# Autodesk Inventor assembly: Butterfly Drive Module_MIR
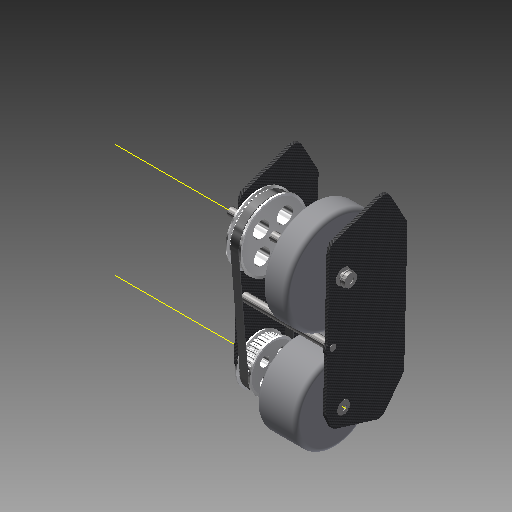
[picture p0: Inventor's stored thumbnail of the model, 512x512]
Saved by Autodesk Inventor 2019.4 (Build 234330000, 330)
## iProperties
Created: 2019-10-18
Part Number: Butterfly Drive Module_MIR
Document SubType Name: Assembly
Designer: admin
Author: admin
## Documents named in this file (10)
- C:\Users\admin\Desktop\FRC 2020 Engineering\GitHub\7738-CAD-prep\Butterfly drive\Butterfly Drive Module_MIR.iam
- C:\Users\admin\Desktop\FRC 2020 Engineering\GitHub\7738-CAD-prep\Butterfly drive\100mm Mecanum StandIn_MIR.ipt
- C:\Users\admin\Desktop\FRC 2020 Engineering\GitHub\7738-CAD-prep\Butterfly drive\100mm Traction Wheel StandIn_MIR.ipt
- C:\Users\admin\Desktop\FRC 2020 Engineering\GitHub\7738-CAD-prep\Butterfly drive\Butterfly Drive Module\Design Accelerator\Synchronous Belts Transmission3_MIR.iam
- C:\Users\admin\Desktop\FRC 2020 Engineering\GitHub\7738-CAD-prep\Butterfly drive\F688ZZ 8mm ID Flange_MIR.ipt
- C:\Users\admin\Desktop\FRC 2020 Engineering\GitHub\7738-CAD-prep\Butterfly drive\F6800Z 10mm ID Flange_MIR.ipt
- C:\Users\admin\Desktop\FRC 2020 Engineering\GitHub\7738-CAD-prep\Butterfly drive\Mecanum Axle_MIR.ipt
- C:\Users\admin\Desktop\FRC 2020 Engineering\GitHub\7738-CAD-prep\Butterfly drive\Motor Axle_MIR.ipt
- C:\Users\admin\Desktop\FRC 2020 Engineering\GitHub\7738-CAD-prep\Butterfly drive\Module Plate 1_MIR.ipt
- C:\Users\admin\Desktop\FRC 2020 Engineering\GitHub\7738-CAD-prep\Butterfly drive\Module Pneumatic Axle_MIR.ipt
## Components (13 placed, 9 different names)
1. 100mm Mecanum StandIn_MIR:1 — Flush:1, Angle:1, Mate:7, Mate:5, Mate:13, Mate:8, Mate:16
2. 100mm Traction Wheel StandIn_MIR:1 — Flush:1, Mate:4, Mate:6, Mate:14
3. Synchronous Belts Transmission3_MIR:1 [sub-assembly] — Mate:7, Mate:6, Mate:5, Mate:10, Mate:9, Mate:15
4. F688ZZ 8mm ID Flange_MIR:1 — Mate:13, Mate:8, Flush:2, Mate:17, Mate:22, Mate:21
5. F688ZZ 8mm ID Flange_MIR:2 — Mate:10, Mate:9, Flush:3, Mate:26, Mate:24
6. F6800Z 10mm ID Flange_MIR:1 — Flush:2, Mate:14, Flush:4, Mate:18
7. F6800Z 10mm ID Flange_MIR:2 — Flush:3, Mate:15
8. Mecanum Axle_MIR:1 — Mate:17, Mate:16
9. F688ZZ 8mm ID Flange_MIR:3 — Flush:4, Mate:18, Mate:20, Mate:19
10. Motor Axle_MIR:1 — Mate:20, Mate:19
11. Module Plate 1_MIR:1 — Mate:23, Mate:22, Mate:21, Mate:29
12. Module Plate 1_MIR:2 — Mate:26, Mate:25, Mate:24, Mate:30
13. Module Pneumatic Axle_MIR:1 — Mate:30, Mate:29
## Relationships (28: Mate 23, Flush 4, Angle 1)
- Flush:1: 100mm Mecanum StandIn_MIR:1 ↔ 100mm Traction Wheel StandIn_MIR:1
- Mate:4: 100mm Traction Wheel StandIn_MIR:1
- Angle:1 (-90 deg): 100mm Mecanum StandIn_MIR:1
- Mate:7 (2 mm): 100mm Mecanum StandIn_MIR:1 ↔ Synchronous Belts Transmission3_MIR:1
- Mate:6: 100mm Traction Wheel StandIn_MIR:1 ↔ Synchronous Belts Transmission3_MIR:1
- Mate:5: 100mm Mecanum StandIn_MIR:1 ↔ Synchronous Belts Transmission3_MIR:1
- Mate:13 (5 mm): 100mm Mecanum StandIn_MIR:1 ↔ F688ZZ 8mm ID Flange_MIR:1
- Mate:8: 100mm Mecanum StandIn_MIR:1 ↔ F688ZZ 8mm ID Flange_MIR:1
- Mate:10 (4 mm): Synchronous Belts Transmission3_MIR:1 ↔ F688ZZ 8mm ID Flange_MIR:2
- Mate:9: Synchronous Belts Transmission3_MIR:1 ↔ F688ZZ 8mm ID Flange_MIR:2
- Flush:2: F688ZZ 8mm ID Flange_MIR:1 ↔ F6800Z 10mm ID Flange_MIR:1
- Mate:14: 100mm Traction Wheel StandIn_MIR:1 ↔ F6800Z 10mm ID Flange_MIR:1
- Flush:3: F688ZZ 8mm ID Flange_MIR:2 ↔ F6800Z 10mm ID Flange_MIR:2
- Mate:15: Synchronous Belts Transmission3_MIR:1 ↔ F6800Z 10mm ID Flange_MIR:2
- Mate:17 (0.3 mm): F688ZZ 8mm ID Flange_MIR:1 ↔ Mecanum Axle_MIR:1
- Mate:16: 100mm Mecanum StandIn_MIR:1 ↔ Mecanum Axle_MIR:1
- Flush:4 (-9.3 mm): F6800Z 10mm ID Flange_MIR:1 ↔ F688ZZ 8mm ID Flange_MIR:3
- Mate:18: F6800Z 10mm ID Flange_MIR:1 ↔ F688ZZ 8mm ID Flange_MIR:3
- Mate:20: F688ZZ 8mm ID Flange_MIR:3 ↔ Motor Axle_MIR:1
- Mate:19 (0.3 mm): F688ZZ 8mm ID Flange_MIR:3 ↔ Motor Axle_MIR:1
- Mate:23: Module Plate 1_MIR:1
- Mate:22 (0.3 mm): F688ZZ 8mm ID Flange_MIR:1 ↔ Module Plate 1_MIR:1
- Mate:21: F688ZZ 8mm ID Flange_MIR:1 ↔ Module Plate 1_MIR:1
- Mate:26 (0.3 mm): F688ZZ 8mm ID Flange_MIR:2 ↔ Module Plate 1_MIR:2
- Mate:25: Module Plate 1_MIR:2
- Mate:24: F688ZZ 8mm ID Flange_MIR:2 ↔ Module Plate 1_MIR:2
- Mate:30: Module Plate 1_MIR:2 ↔ Module Pneumatic Axle_MIR:1
- Mate:29 (0.3 mm): Module Plate 1_MIR:1 ↔ Module Pneumatic Axle_MIR:1
